# Autodesk Inventor assembly: Correct
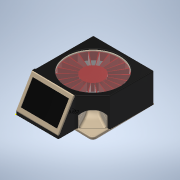
[picture p0: Inventor's stored thumbnail of the model, 180x180]
Saved by Autodesk Inventor 2022 (Build 260153000, 153)
## iProperties
Created: 2023-02-27
Part Number: Correct
Document SubType Name: Assembly
Designer: zarek
Author: zarek
## Documents named in this file (16)
- C:\Users\zarek\OneDrive\Desktop\Random New Stuff\SPB\Overall Fancy.iam
- C:\Users\zarek\OneDrive\Desktop\Random New Stuff\SPB\Capsule_Design_Final.ipt
- C:\Users\zarek\OneDrive\Desktop\Random New Stuff\SPB\Motor_Key.ipt
- C:\Users\zarek\OneDrive\Desktop\Random New Stuff\SPB\GrabCad Parts\Stepper 28BYJ48.ipt
- C:\Users\zarek\OneDrive\Desktop\Random New Stuff\SPB\Drop_Plate.ipt
- C:\Users\zarek\OneDrive\Desktop\Random New Stuff\SPB\Box_Walls_2.ipt
- C:\Users\zarek\OneDrive\Desktop\Random New Stuff\SPB\Lid Parts\Lid Assembly.iam
- C:\Users\zarek\OneDrive\Desktop\Random New Stuff\SPB\Servo&Holder.iam
- C:\Users\zarek\OneDrive\Desktop\Random New Stuff\SPB\Hook.ipt
- C:\Users\zarek\OneDrive\Desktop\Random New Stuff\SPB\Lid_Inside_Base.ipt
- C:\Users\zarek\OneDrive\Desktop\Random New Stuff\SPB\TouchScreen Housing\Touch Screen Assembly_2.iam
- C:\Users\zarek\OneDrive\Desktop\Random New Stuff\SPB\Base_Plate_Assembly.iam
- C:\Users\zarek\OneDrive\Desktop\Random New Stuff\SPB\Slide.ipt
- C:\Users\zarek\OneDrive\Desktop\Random New Stuff\SPB\GrabCad Parts\Raspberry Pi 4 Model B.ipt
- C:\Users\zarek\OneDrive\Desktop\Random New Stuff\SPB\GrabCad Parts\LED 5mm.ipt
- C:\Users\zarek\Downloads\ULN2003 Stepper Driver.ipt
## Components (15 placed, 15 different names)
1. Capsule_Design_Final:1 — Rotational:2
2. Motor_Key:1 — Rotational:1, Rotational:2
3. Stepper 28BYJ48:1 — Rotational:1, Slider:3
4. Drop_Plate:1
5. Box_Walls_2:1 — Rotational:5, Flush:1, Flush:2
6. Lid Assembly:1 [sub-assembly] — Flush:1, Flush:2
7. Servo&Holder:1 [sub-assembly] — Rotational:3
8. Hook:1 — Rotational:3
9. Lid_Inside_Base:1
10. Touch Screen Assembly_2:1 [sub-assembly]
11. Base_Plate_Assembly:1 [sub-assembly] — Slider:3, Mate:1, Mate:2, Rotational:4, Rotational:5
12. Slide:1 — Mate:1, Mate:2
13. Raspberry Pi 4 Model B:1
14. LED 5mm:1 — Rotational:4
15. ULN2003 Stepper Driver:1
## Relationships (10: RevoluteJoint 5, Mate 2, Flush 2, TranslationJoint 1)
- Rotational:1 [RevoluteJoint]: Motor_Key:1 ↔ Stepper 28BYJ48:1
- Rotational:2 [RevoluteJoint] (1 mm): Capsule_Design_Final:1 ↔ Motor_Key:1
- Rotational:3 [RevoluteJoint]: Servo&Holder:1 ↔ Hook:1
- Slider:3 [TranslationJoint]: Stepper 28BYJ48:1 ↔ Base_Plate_Assembly:1
- Mate:1: Base_Plate_Assembly:1 ↔ Slide:1
- Mate:2: Base_Plate_Assembly:1 ↔ Slide:1
- Rotational:4 [RevoluteJoint]: Base_Plate_Assembly:1 ↔ LED 5mm:1
- Rotational:5 [RevoluteJoint]: Box_Walls_2:1 ↔ Base_Plate_Assembly:1
- Flush:1: Box_Walls_2:1 ↔ Lid Assembly:1
- Flush:2: Box_Walls_2:1 ↔ Lid Assembly:1
